# Autodesk Inventor assembly: TestAssembly
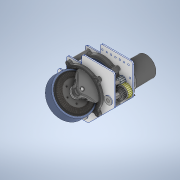
[picture p0: Inventor's stored thumbnail of the model, 180x180]
Saved by Autodesk Inventor 2020 (Build 240168000, 168)
## iProperties
Created: 2019-05-09
Part Number: TestAssembly
Document SubType Name: Assembly
Designer: Connor
Author: Connor
## Documents named in this file (30)
- C:\Users\glesl\Documents\FRC 2019\Grab cad\Swerve\TorqyoDrift\TestAssembly.iam
- C:\Users\glesl\Documents\FRC 2019\Grab cad\Imported Components\Wheels and Hubs\VEX Traction Wheels\TractionWheel 4x1\TractionWheel 4x1.iam
- C:\Users\glesl\Documents\FRC 2019\Grab cad\Swerve\TorqyoDrift\15t_bevel.ipt
- C:\Users\glesl\Documents\FRC 2019\Grab cad\Swerve\TorqyoDrift\60t_bevel.ipt
- C:\Users\glesl\Documents\FRC 2019\Grab cad\Swerve\TorqyoDrift\ImportedComponentsPlus\Bearings\SA035XPO.ipt
- C:\Users\glesl\Documents\FRC 2019\Grab cad\Swerve\TorqyoDrift\ImportedComponentsPlus\Hex Gears\16t_Aluminum_Spur_Gear_20_DP_3_8_Hex_Bore_217-5450.ipt
- C:\Users\glesl\Documents\FRC 2019\Grab cad\Imported Components\Bearings\Radial_0.25x0.375x0.125.ipt
- C:\Users\glesl\Documents\FRC 2019\Grab cad\Swerve\TorqyoDrift\DriveShaft.ipt
- C:\Users\glesl\Documents\FRC 2019\Grab cad\Imported Components\Bearings\Radial_0.25x0.5x0.188.ipt
- C:\Users\glesl\Documents\FRC 2019\Grab cad\Swerve\TorqyoDrift\SplitBracketHead.ipt
- C:\Users\glesl\Documents\FRC 2019\Grab cad\Swerve\TorqyoDrift\BlueTreadMax.ipt
- C:\Users\glesl\Documents\FRC 2019\Grab cad\Swerve\TorqyoDrift\SplitBracketNut.ipt
- C:\Users\glesl\Documents\FRC 2019\Grab cad\Swerve\TorqyoDrift\ImportedComponentsPlus\91259A723_ALLOY STEEL SHOULDER SCREW.ipt
- C:\Users\glesl\Documents\FRC 2019\Grab cad\Swerve\TorqyoDrift\CenterColumnV2.ipt
- C:\Users\glesl\Documents\FRC 2019\Grab cad\Swerve\TorqyoDrift\AlternateRingGearAssembly.iam
- C:\Users\glesl\Documents\FRC 2019\Grab cad\Swerve\TorqyoDrift\BearingClamp.ipt
- C:\Users\glesl\Documents\FRC 2019\Grab cad\Swerve\TorqyoDrift\ImportedComponentsPlus\Bearings\0_500_ID_x_1_125_OD_x_0_313_WD_Flanged_Bearing_217-2731 (1).ipt
- C:\Users\glesl\Documents\FRC 2019\Grab cad\Swerve\TorqyoDrift\BottomPlate.ipt
- C:\Users\glesl\Documents\FRC 2019\Grab cad\Swerve\TorqyoDrift\ImportedComponentsPlus\REV-21-1650.ipt
- C:\Users\glesl\Documents\FRC 2019\Grab cad\Swerve\TorqyoDrift\BearingCage.ipt
- C:\Users\glesl\Documents\FRC 2019\Grab cad\Swerve\TorqyoDrift\TopPlate.ipt
- C:\Users\glesl\Documents\FRC 2019\Grab cad\Swerve\TorqyoDrift\ImportedComponentsPlus\Motor Pinions\12t_Aluminum_Spur_Gear_20_DP_CIM_Motor_217-2614.ipt
- C:\Users\glesl\Documents\FRC 2019\Grab cad\Swerve\TorqyoDrift\ImportedComponentsPlus\Timing Pulleys\18t_x_9mm_Wide_Double_Flange_Aluminum_Pulley_HTD_5mm_1_2_Hex_Bore_217-3225.ipt
- C:\Users\glesl\Documents\FRC 2019\Grab cad\Swerve\TorqyoDrift\MotorBracket.ipt
- C:\Users\glesl\Documents\FRC 2019\Grab cad\Swerve\TorqyoDrift\GearShaft.ipt
- C:\Users\glesl\Documents\FRC 2019\Grab cad\Swerve\TorqyoDrift\ImportedComponentsPlus\Bearings\0_375_ID_x_0_875_OD_x_0_281_WD_Radial_Bearing_217-3239.ipt
- C:\Users\glesl\Documents\FRC 2019\Grab cad\Swerve\TorqyoDrift\ImportedComponentsPlus\Bearings\0_375_ID_x_0_875_OD_x_0_280_WD_Flanged_Bearing_217-2733.ipt
- C:\Users\glesl\Documents\FRC 2019\Grab cad\Swerve\TorqyoDrift\ImportedComponentsPlus\Hex Gears\24t_Steel_Spur_Gear_20_DP_1_2_Hex_Bore_217-5464.ipt
- C:\Users\glesl\Documents\FRC 2019\Grab cad\Swerve\TorqyoDrift\ButterflyEncoderBracket.ipt
- C:\Users\glesl\Documents\FRC 2019\Grab cad\Swerve\TorqyoDrift\ImportedComponentsPlus\Sensors\TT_Electronics_Encoder_6127V1A360L.5FS.ipt
## Components (45 placed, 29 different names)
1. TractionWheel 4x1:1 [sub-assembly] — Mate:1, Mate:2, Mate:3, Mate:4, Mate:5, Mate:6, Mate:51, Mate:52, Mate:54, Mate:57
2. 15t_bevel:1 — Tangent:1, Flush:1, Mate:7, Mate:30, Mate:31, Angle:3
3. 60t_bevel:1 — Mate:4, Mate:5, Mate:6, Tangent:1, Flush:1, Mate:7, Insert:8
4. 15t_bevel:2 — Tangent:2, Mate:9, Flush:2, Mate:32, Angle:4, Angle:5, Mate:56
5. 60t_bevel:2 — Mate:1, Mate:2, Mate:3, Tangent:2, Mate:9, Flush:2, Insert:7
6. SA035XPO:1 — Mate:49, Mate:50, Mate:55, Mate:60, Mate:61, Insert:6, Insert:9
7. 16t_Aluminum_Spur_Gear_20_DP_3_8_Hex_Bore_217-5450:1 — Mate:30, Mate:31, Angle:3, Flush:3
8. 16t_Aluminum_Spur_Gear_20_DP_3_8_Hex_Bore_217-5450:2 — Mate:32, Angle:4, Flush:4
9. Radial_0.25x0.375x0.125:1 — Insert:2
10. Radial_0.25x0.375x0.125:2 — Insert:1
11. DriveShaft:1 — Insert:4
12. Radial_0.25x0.5x0.188:1 — Mate:46, Mate:47, Insert:3
13. Radial_0.25x0.5x0.188:2 — Insert:4, Insert:5
14. DriveShaft:2 — Mate:46, Mate:47
15. SplitBracketHead:1 — Angle:5, Mate:49, Mate:50, Mate:56, Mate:57, Mate:58, Mate:59, Insert:1, Mate:68
16. BlueTreadMax:1 — Mate:51, Mate:52
17. SplitBracketNut:1 — Mate:54, Mate:55, Insert:2
18. 91259A723_ALLOY STEEL SHOULDER SCREW:1 — Mate:58, Mate:59
19. CenterColumnV2:1 — Mate:60, Mate:61, Mate:62, Mate:63, Insert:3, Insert:5, Mate:68, Mate:129, Mate:130, Mate:131
20. AlternateRingGearAssembly:1 [sub-assembly] — Mate:63, Mate:64, Flush:4, Flush:5
21. AlternateRingGearAssembly:2 [sub-assembly] — Mate:62, Flush:3, Mate:64, Flush:8
22. BearingClamp:1 — Insert:6, Mate:69
23. 0_500_ID_x_1_125_OD_x_0_313_WD_Flanged_Bearing_217-2731 (1):1 — Insert:7
24. 0_500_ID_x_1_125_OD_x_0_313_WD_Flanged_Bearing_217-2731 (1):2 — Insert:8
25. BottomPlate:2 — Insert:9, Mate:72, Mate:81, Mate:83, Insert:16, Insert:17
26. BearingCage:1 — Mate:69, Mate:71, Mate:72, Mate:80, Mate:81, Mate:82, Mate:83
27. TopPlate:1 — Mate:71, Mate:80, Mate:82, Mate:84, Mate:85, Mate:86, Mate:87, Mate:88, Mate:89, Mate:98, Mate:105, Mate:108, Flush:16, Mate:109, Flush:17, Mate:126, Mate:127, Mate:128
28. REV-21-1650:1 — Insert:15, Mate:91, Mate:92, Mate:95
29. REV-21-1650:2 — Insert:14, Mate:93, Mate:94, Mate:104
30. 12t_Aluminum_Spur_Gear_20_DP_CIM_Motor_217-2614:1 — Insert:14
31. 12t_Aluminum_Spur_Gear_20_DP_CIM_Motor_217-2614:2 — Insert:15, Flush:18
32. 18t_x_9mm_Wide_Double_Flange_Aluminum_Pulley_HTD_5mm_1_2_Hex_Bore_217-3225:2 — Flush:5, Mate:105, Mate:110, Mate:111
33. 18t_x_9mm_Wide_Double_Flange_Aluminum_Pulley_HTD_5mm_1_2_Hex_Bore_217-3225:3 — Flush:8, Mate:98, Mate:112
34. MotorBracket:1 — Mate:87, Mate:88, Mate:89, Mate:93, Mate:94, Mate:104
35. MotorBracket:2 — Mate:84, Mate:85, Mate:86, Mate:91, Mate:92, Mate:95
36. GearShaft:1 — Insert:19
37. GearShaft:2 — Insert:18
38. 0_375_ID_x_0_875_OD_x_0_281_WD_Radial_Bearing_217-3239:1 — Mate:108, Flush:16
39. 0_375_ID_x_0_875_OD_x_0_281_WD_Radial_Bearing_217-3239:2 — Mate:109, Flush:17
40. 0_375_ID_x_0_875_OD_x_0_280_WD_Flanged_Bearing_217-2733:1 — Insert:16, Insert:18
41. 0_375_ID_x_0_875_OD_x_0_280_WD_Flanged_Bearing_217-2733:2 — Insert:17, Insert:19
42. 24t_Steel_Spur_Gear_20_DP_1_2_Hex_Bore_217-5464:1 — Mate:110, Mate:111
43. 24t_Steel_Spur_Gear_20_DP_1_2_Hex_Bore_217-5464:2 — Mate:112, Flush:18
44. ButterflyEncoderBracket:1 — Angle:8, Mate:129, Mate:130, Mate:131
45. TT_Electronics_Encoder_6127V1A360L.5FS:1 — Mate:126, Mate:127, Mate:128, Angle:8
## Relationships (91: Mate 61, Insert 15, Flush 9, Angle 4, Tangent 2)
- Mate:1: TractionWheel 4x1:1 ↔ 60t_bevel:2
- Mate:2: TractionWheel 4x1:1 ↔ 60t_bevel:2
- Mate:3: TractionWheel 4x1:1 ↔ 60t_bevel:2
- Mate:4: TractionWheel 4x1:1 ↔ 60t_bevel:1
- Mate:5: TractionWheel 4x1:1 ↔ 60t_bevel:1
- Mate:6: TractionWheel 4x1:1 ↔ 60t_bevel:1
- Tangent:1 (2 mm): 15t_bevel:1 ↔ 60t_bevel:1
- Flush:1 (56 mm): 15t_bevel:1 ↔ 60t_bevel:1
- Mate:7: 15t_bevel:1 ↔ 60t_bevel:1
- Tangent:2 (2 mm): 15t_bevel:2 ↔ 60t_bevel:2
- Mate:9 (-56 mm): 15t_bevel:2 ↔ 60t_bevel:2
- Flush:2: 15t_bevel:2 ↔ 60t_bevel:2
- Mate:30: 15t_bevel:1 ↔ 16t_Aluminum_Spur_Gear_20_DP_3_8_Hex_Bore_217-5450:1
- Mate:31: 15t_bevel:1 ↔ 16t_Aluminum_Spur_Gear_20_DP_3_8_Hex_Bore_217-5450:1
- Angle:3 (0 deg): 15t_bevel:1 ↔ 16t_Aluminum_Spur_Gear_20_DP_3_8_Hex_Bore_217-5450:1
- Mate:32: 15t_bevel:2 ↔ 16t_Aluminum_Spur_Gear_20_DP_3_8_Hex_Bore_217-5450:2
- Angle:4 (0 deg): 15t_bevel:2 ↔ 16t_Aluminum_Spur_Gear_20_DP_3_8_Hex_Bore_217-5450:2
- Mate:46: Radial_0.25x0.5x0.188:1 ↔ DriveShaft:2
- Mate:47: Radial_0.25x0.5x0.188:1 ↔ DriveShaft:2
- Angle:5 (0 deg): 15t_bevel:2 ↔ SplitBracketHead:1
- Mate:49: SA035XPO:1 ↔ SplitBracketHead:1
- Mate:50: SA035XPO:1 ↔ SplitBracketHead:1
- Mate:51: TractionWheel 4x1:1 ↔ BlueTreadMax:1
- Mate:52: TractionWheel 4x1:1 ↔ BlueTreadMax:1
- Mate:54: TractionWheel 4x1:1 ↔ SplitBracketNut:1
- Mate:55: SA035XPO:1 ↔ SplitBracketNut:1
- Mate:56: 15t_bevel:2 ↔ SplitBracketHead:1
- Mate:57: TractionWheel 4x1:1 ↔ SplitBracketHead:1
- Mate:58: SplitBracketHead:1 ↔ 91259A723_ALLOY STEEL SHOULDER SCREW:1
- Mate:59: SplitBracketHead:1 ↔ 91259A723_ALLOY STEEL SHOULDER SCREW:1
- Insert:1: Radial_0.25x0.375x0.125:2 ↔ SplitBracketHead:1
- Insert:2: Radial_0.25x0.375x0.125:1 ↔ SplitBracketNut:1
- Mate:60: SA035XPO:1 ↔ CenterColumnV2:1
- Mate:61: SA035XPO:1 ↔ CenterColumnV2:1
- Mate:62: CenterColumnV2:1 ↔ AlternateRingGearAssembly:2
- Flush:3: 16t_Aluminum_Spur_Gear_20_DP_3_8_Hex_Bore_217-5450:1 ↔ AlternateRingGearAssembly:2
- Mate:63: CenterColumnV2:1 ↔ AlternateRingGearAssembly:1
- Mate:64 (1.016 mm): AlternateRingGearAssembly:1 ↔ AlternateRingGearAssembly:2
- Flush:4: 16t_Aluminum_Spur_Gear_20_DP_3_8_Hex_Bore_217-5450:2 ↔ AlternateRingGearAssembly:1
- Insert:3: Radial_0.25x0.5x0.188:1 ↔ CenterColumnV2:1
- Insert:4: DriveShaft:1 ↔ Radial_0.25x0.5x0.188:2
- Insert:5: Radial_0.25x0.5x0.188:2 ↔ CenterColumnV2:1
- Insert:6: SA035XPO:1 ↔ BearingClamp:1
- Insert:7: 60t_bevel:2 ↔ 0_500_ID_x_1_125_OD_x_0_313_WD_Flanged_Bearing_217-2731 (1):1
- Insert:8: 60t_bevel:1 ↔ 0_500_ID_x_1_125_OD_x_0_313_WD_Flanged_Bearing_217-2731 (1):2
- Insert:9: SA035XPO:1 ↔ BottomPlate:2
- Mate:68: SplitBracketHead:1 ↔ CenterColumnV2:1
- Mate:69: BearingClamp:1 ↔ BearingCage:1
- Mate:71: BearingCage:1 ↔ TopPlate:1
- Mate:72: BottomPlate:2 ↔ BearingCage:1
- Insert:14: REV-21-1650:2 ↔ 12t_Aluminum_Spur_Gear_20_DP_CIM_Motor_217-2614:1
- Flush:5 (0.4699 mm): AlternateRingGearAssembly:1 ↔ 18t_x_9mm_Wide_Double_Flange_Aluminum_Pulley_HTD_5mm_1_2_Hex_Bore_217-3225:2
- Mate:80: BearingCage:1 ↔ TopPlate:1
- Mate:81: BottomPlate:2 ↔ BearingCage:1
- Mate:82: BearingCage:1 ↔ TopPlate:1
- Mate:83: BottomPlate:2 ↔ BearingCage:1
- Insert:15: REV-21-1650:1 ↔ 12t_Aluminum_Spur_Gear_20_DP_CIM_Motor_217-2614:2
- Flush:8 (0.4826 mm): AlternateRingGearAssembly:2 ↔ 18t_x_9mm_Wide_Double_Flange_Aluminum_Pulley_HTD_5mm_1_2_Hex_Bore_217-3225:3
- Mate:84: TopPlate:1 ↔ MotorBracket:2
- Mate:85: TopPlate:1 ↔ MotorBracket:2
- Mate:86: TopPlate:1 ↔ MotorBracket:2
- Mate:87: TopPlate:1 ↔ MotorBracket:1
- Mate:88: TopPlate:1 ↔ MotorBracket:1
- Mate:89: TopPlate:1 ↔ MotorBracket:1
- Mate:91: REV-21-1650:1 ↔ MotorBracket:2
- Mate:92: REV-21-1650:1 ↔ MotorBracket:2
- Mate:93: REV-21-1650:2 ↔ MotorBracket:1
- Mate:94: REV-21-1650:2 ↔ MotorBracket:1
- Mate:95: REV-21-1650:1 ↔ MotorBracket:2
- Mate:98: TopPlate:1 ↔ 18t_x_9mm_Wide_Double_Flange_Aluminum_Pulley_HTD_5mm_1_2_Hex_Bore_217-3225:3
- Mate:104: REV-21-1650:2 ↔ MotorBracket:1
- Mate:105: TopPlate:1 ↔ 18t_x_9mm_Wide_Double_Flange_Aluminum_Pulley_HTD_5mm_1_2_Hex_Bore_217-3225:2
- Mate:108: TopPlate:1 ↔ 0_375_ID_x_0_875_OD_x_0_281_WD_Radial_Bearing_217-3239:1
- Flush:16: TopPlate:1 ↔ 0_375_ID_x_0_875_OD_x_0_281_WD_Radial_Bearing_217-3239:1
- Mate:109: TopPlate:1 ↔ 0_375_ID_x_0_875_OD_x_0_281_WD_Radial_Bearing_217-3239:2
- Flush:17: TopPlate:1 ↔ 0_375_ID_x_0_875_OD_x_0_281_WD_Radial_Bearing_217-3239:2
- Insert:16: BottomPlate:2 ↔ 0_375_ID_x_0_875_OD_x_0_280_WD_Flanged_Bearing_217-2733:1
- Insert:17: BottomPlate:2 ↔ 0_375_ID_x_0_875_OD_x_0_280_WD_Flanged_Bearing_217-2733:2
- Insert:18: GearShaft:2 ↔ 0_375_ID_x_0_875_OD_x_0_280_WD_Flanged_Bearing_217-2733:1
- Insert:19: GearShaft:1 ↔ 0_375_ID_x_0_875_OD_x_0_280_WD_Flanged_Bearing_217-2733:2
- Mate:110: 18t_x_9mm_Wide_Double_Flange_Aluminum_Pulley_HTD_5mm_1_2_Hex_Bore_217-3225:2 ↔ 24t_Steel_Spur_Gear_20_DP_1_2_Hex_Bore_217-5464:1
- Mate:111: 18t_x_9mm_Wide_Double_Flange_Aluminum_Pulley_HTD_5mm_1_2_Hex_Bore_217-3225:2 ↔ 24t_Steel_Spur_Gear_20_DP_1_2_Hex_Bore_217-5464:1
- Mate:112: 18t_x_9mm_Wide_Double_Flange_Aluminum_Pulley_HTD_5mm_1_2_Hex_Bore_217-3225:3 ↔ 24t_Steel_Spur_Gear_20_DP_1_2_Hex_Bore_217-5464:2
- Flush:18: 12t_Aluminum_Spur_Gear_20_DP_CIM_Motor_217-2614:2 ↔ 24t_Steel_Spur_Gear_20_DP_1_2_Hex_Bore_217-5464:2
- Mate:126: TopPlate:1 ↔ TT_Electronics_Encoder_6127V1A360L.5FS:1
- Mate:127: TopPlate:1 ↔ TT_Electronics_Encoder_6127V1A360L.5FS:1
- Mate:128: TopPlate:1 ↔ TT_Electronics_Encoder_6127V1A360L.5FS:1
- Angle:8 (0 deg): ButterflyEncoderBracket:1 ↔ TT_Electronics_Encoder_6127V1A360L.5FS:1
- Mate:129: CenterColumnV2:1 ↔ ButterflyEncoderBracket:1
- Mate:130: CenterColumnV2:1 ↔ ButterflyEncoderBracket:1
- Mate:131: CenterColumnV2:1 ↔ ButterflyEncoderBracket:1
